# Autodesk Inventor assembly: Ensamblaje de respuesto
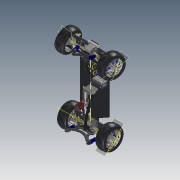
[picture p0: Inventor's stored thumbnail of the model, 180x180]
Saved by Autodesk Inventor 2015 (Build 190159000, 159)
## iProperties
Created: 2015-12-07
Part Number: Ensamblaje de respuesto
Document SubType Name: Assembly
Designer: MIGUEL ANGEL
Author: MIGUEL ANGEL
## Documents named in this file (59)
- C:\Users\MIGUEL ANGEL\Desktop\COCHE\Ensamblaje de respuesto.iam
- C:\Users\MIGUEL ANGEL\Desktop\COCHE\chasis.ipt
- C:\Users\MIGUEL ANGEL\Desktop\COCHE\estructura para ejes ruedas.ipt
- C:\Users\MIGUEL ANGEL\Desktop\COCHE\Pieza direccion.ipt
- C:\Users\MIGUEL ANGEL\Desktop\COCHE\pieza 2 direccion.ipt
- C:\Users\MIGUEL ANGEL\Desktop\COCHE\pieza de chasis.ipt
- C:\Users\MIGUEL ANGEL\Desktop\COCHE\pieza plastico.ipt
- C:\Users\MIGUEL ANGEL\Desktop\COCHE\rotula-eje.ipt
- C:\Users\MIGUEL ANGEL\Desktop\COCHE\pivote de dirección 1.iam
- C:\Users\MIGUEL ANGEL\Desktop\COCHE\tapeta.ipt
- C:\Users\MIGUEL ANGEL\Desktop\COCHE\pieza eje rueda.ipt
- C:\Users\MIGUEL ANGEL\Desktop\COCHE\caja parte 1.ipt
- C:\Users\MIGUEL ANGEL\Desktop\COCHE\pieza del eje.ipt
- C:\Users\MIGUEL ANGEL\Desktop\COCHE\caja de direccion\caja de direccion.iam
- C:\Users\MIGUEL ANGEL\Desktop\COCHE\barra con agarraderas.iam
- C:\Users\MIGUEL ANGEL\Desktop\COCHE\placa direccion 2.ipt
- C:\Users\MIGUEL ANGEL\Desktop\COCHE\pieza articulada de uniones.ipt
- C:\Users\MIGUEL ANGEL\Desktop\COCHE\Ensamblaje de respuesto\Design Accelerator\Conexión por perno1.iam
- C:\Users\MIGUEL ANGEL\Desktop\COCHE\Ensamblaje de respuesto\Design Accelerator\Conexión por perno2.iam
- C:\Users\MIGUEL ANGEL\Desktop\COCHE\barra con agarraderas pequeña.iam
- C:\Users\MIGUEL ANGEL\Desktop\COCHE\eje rueda bueno.ipt
- C:\Users\MIGUEL ANGEL\Desktop\COCHE\tubo para hueso.ipt
- C:\Users\MIGUEL ANGEL\Desktop\COCHE\pieza direccion placa.ipt
- C:\Users\MIGUEL ANGEL\Desktop\COCHE\prueba engranajes.iam
- C:\Users\MIGUEL ANGEL\Desktop\COCHE\eje principal 8 diametro.ipt
- C:\Users\MIGUEL ANGEL\Desktop\COCHE\pieza parte delantera.ipt
- C:\Users\MIGUEL ANGEL\Desktop\COCHE\conexion entre amortiguador y placa.ipt
- C:\Users\MIGUEL ANGEL\Desktop\COCHE\pieza direccion trasera.ipt
- C:\Users\MIGUEL ANGEL\Desktop\COCHE\soporte eje.ipt
- C:\Users\MIGUEL ANGEL\Desktop\COCHE\motor.ipt
- C:\Users\MIGUEL ANGEL\Desktop\COCHE\engranaje 2.iam
- C:\Users\MIGUEL ANGEL\Desktop\COCHE\engranaje 1.iam
- C:\Users\MIGUEL ANGEL\Desktop\COCHE\agarraderas.iam
- C:\Users\MIGUEL ANGEL\Desktop\COCHE\NORMALIZADAS\es-ES\DIN 835\DIN 835 - M6 x 25 - 1.ipt
- C:\Users\MIGUEL ANGEL\Desktop\COCHE\NORMALIZADAS\es-ES\DIN 439-2\DIN 439 - M6 x 1.ipt
- C:\Users\MIGUEL ANGEL\Desktop\COCHE\NORMALIZADAS\es-ES\ANSI B18.22 M\ANSI B18.22M - 6 N.ipt
- C:\Users\MIGUEL ANGEL\Desktop\COCHE\eje rueda bueno trasero.ipt
- C:\Users\MIGUEL ANGEL\Desktop\COCHE\pieza parte trasera.ipt
- C:\Users\MIGUEL ANGEL\Desktop\COCHE\amortiguador.iam
- C:\Users\MIGUEL ANGEL\Desktop\COCHE\armadura.ipt
- C:\Users\MIGUEL ANGEL\Desktop\COCHE\La LLanta.ipt
- C:\Users\MIGUEL ANGEL\Desktop\COCHE\el nuematico.ipt
- C:\Users\MIGUEL ANGEL\Desktop\COCHE\parte motor 2.ipt
- C:\Users\MIGUEL ANGEL\Desktop\COCHE\parte motor 3.ipt
- C:\Users\MIGUEL ANGEL\Desktop\COCHE\caja parte 2 buena.ipt
- C:\Users\MIGUEL ANGEL\Desktop\COCHE\Ensamblaje de respuesto\Design Accelerator\Conexión por perno3.iam
- C:\Users\MIGUEL ANGEL\Desktop\COCHE\Ensamblaje de respuesto\Design Accelerator\Conexión por perno4.iam
- C:\Users\MIGUEL ANGEL\Desktop\COCHE\Ensamblaje de respuesto\Design Accelerator\Conexión por perno5.iam
- C:\Users\MIGUEL ANGEL\Desktop\COCHE\Ensamblaje de respuesto\Design Accelerator\Conexión por perno6.iam
- C:\Users\MIGUEL ANGEL\Desktop\COCHE\Ensamblaje de respuesto\Design Accelerator\Conexión por perno7.iam
- C:\Users\MIGUEL ANGEL\Desktop\COCHE\Ensamblaje de respuesto\Design Accelerator\Conexión por perno8.iam
- C:\Users\MIGUEL ANGEL\Desktop\COCHE\Ensamblaje de respuesto\Design Accelerator\Conexión por perno9.iam
- C:\Users\MIGUEL ANGEL\Desktop\COCHE\Ensamblaje de respuesto\Design Accelerator\Conexión por perno10.iam
- C:\Users\MIGUEL ANGEL\Desktop\COCHE\Ensamblaje de respuesto\Design Accelerator\Conexión por perno12.iam
- C:\Users\MIGUEL ANGEL\Desktop\COCHE\Ensamblaje de respuesto\Design Accelerator\Conexión por perno13.iam
- C:\Users\MIGUEL ANGEL\Desktop\COCHE\Ensamblaje de respuesto\Design Accelerator\Conexión por perno14.iam
- C:\Users\MIGUEL ANGEL\Desktop\COCHE\Ensamblaje de respuesto\Design Accelerator\Conexión por perno15.iam
- C:\Users\MIGUEL ANGEL\Desktop\COCHE\Ensamblaje de respuesto\Design Accelerator\Conexión por perno17.iam
- C:\Users\MIGUEL ANGEL\Desktop\COCHE\Ensamblaje de respuesto\Design Accelerator\Conexión por perno18.iam
## Components (138 placed, 43 different names)
1. chasis:1 — Coincidencia:5, Nivelación:1, Coincidencia:6, Coincidencia:10, Insertar:3, Insertar:4, Coincidencia:27, Coincidencia:28, Nivelación:6, Coincidencia:58, Coincidencia:59, Coincidencia:60, Coincidencia:87, Coincidencia:88, Coincidencia:89, Coincidencia:95, Coincidencia:96, Coincidencia:97, Coincidencia:140, Coincidencia:141, Coincidencia:142, Ángulo:21, Coincidencia:221, Coincidencia:225, Ángulo:25, Coincidencia:267, Coincidencia:269
2. estructura para ejes ruedas:1 — Coincidencia:7, Coincidencia:8, Coincidencia:11, Coincidencia:108, Coincidencia:109, Coincidencia:209
3. pieza de chasis:1 — Coincidencia:5, Nivelación:1, Coincidencia:6, Coincidencia:7, Insertar:1, Ángulo:1, Coincidencia:16, Insertar:2, Ángulo:2
4. pieza plastico:1 — Insertar:1, Ángulo:1, Coincidencia:8
5. rotula-eje:1 — Nivelación:17, Coincidencia:233, Coincidencia:234, Coincidencia:236
6. pieza de chasis:2 — Coincidencia:10, Coincidencia:11
7. pivote de dirección 1:1 [sub-assembly] — Insertar:3, Coincidencia:54, Coincidencia:55, Insertar:13, Coincidencia:68
8. pivote de dirección 1:2 [sub-assembly] — Insertar:4, Coincidencia:52, Coincidencia:53, Coincidencia:69, Coincidencia:70, Coincidencia:205, Ángulo:25
9. estructura para ejes ruedas:2 — Coincidencia:16, Coincidencia:17, Coincidencia:128, Coincidencia:129, Coincidencia:187
10. pieza plastico:2 — Insertar:2, Ángulo:2, Coincidencia:17
11. rotula-eje:2 — Coincidencia:62, Coincidencia:63, Nivelación:18, Coincidencia:245
12. estructura para ejes ruedas:3 — Coincidencia:29, Coincidencia:32, Coincidencia:33, Coincidencia:79, Coincidencia:80, Coincidencia:215
13. estructura para ejes ruedas:4 — Coincidencia:30, Coincidencia:31, Coincidencia:81, Coincidencia:82, Coincidencia:211, Ángulo:21
14. pieza de chasis:3 — Coincidencia:27, Coincidencia:28, Coincidencia:29, Coincidencia:30, Insertar:6, Insertar:7, Nivelación:6, Coincidencia:32
15. pieza plastico:3 — Insertar:6, Coincidencia:31
16. pieza plastico:4 — Insertar:7, Coincidencia:33
17. caja parte 1:1 — Nivelación:8, Coincidencia:77, Coincidencia:95, Coincidencia:96, Coincidencia:97, Coincidencia:102, Insertar:38, Coincidencia:268, Insertar:52, Coincidencia:283, Coincidencia:284, Coincidencia:285, Coincidencia:286
18. placa direccion 2:1 — Coincidencia:50, Coincidencia:51, Coincidencia:56, Coincidencia:57, Coincidencia:203, Coincidencia:204, Coincidencia:205
19. pieza articulada de uniones:1 — Coincidencia:50, Coincidencia:204, Coincidencia:250
20. pieza articulada de uniones:2 — Coincidencia:51, Coincidencia:203, Coincidencia:249
21. Conexión por perno:1 [sub-assembly] — Coincidencia:52, Coincidencia:53, Coincidencia:57
22. Conexión por perno:2 [sub-assembly] — Coincidencia:54, Coincidencia:55, Coincidencia:56
23. barra con agarraderas pequeña:1 [sub-assembly] — Insertar:13, Insertar:15
24. caja de direccion:1 [sub-assembly] — Coincidencia:58, Coincidencia:59, Coincidencia:60, Insertar:15, Coincidencia:275, Coincidencia:276, Coincidencia:277, Coincidencia:278
25. eje rueda bueno:1 — Coincidencia:62, Coincidencia:63, Coincidencia:246, Nivelación:19, Coincidencia:248
26. pieza direccion placa:1 — Coincidencia:68, Coincidencia:69, Coincidencia:70
27. pieza parte delantera:1 — Nivelación:8, Coincidencia:77, Insertar:21, Insertar:22, Coincidencia:102, Coincidencia:116, Coincidencia:123, Coincidencia:133, Coincidencia:158, Nivelación:12, Coincidencia:161, Coincidencia:220, Coincidencia:260
28. conexion entre amortiguador y placa:1 — Insertar:21, Coincidencia:208
29. conexion entre amortiguador y placa:2 — Insertar:22, Coincidencia:186
30. pieza direccion trasera:1 — Coincidencia:79, Coincidencia:80, Coincidencia:83, Coincidencia:84, Coincidencia:170, Coincidencia:171, Coincidencia:178, Nivelación:14, Coincidencia:181, Coincidencia:182, Coincidencia:217
31. pieza direccion trasera:2 — Coincidencia:81, Coincidencia:82, Coincidencia:85, Coincidencia:86, Coincidencia:167, Coincidencia:168, Coincidencia:173, Nivelación:13, Coincidencia:176, Coincidencia:177, Coincidencia:219
32. rotula-eje:3 — Coincidencia:83, Coincidencia:84, Coincidencia:147, Coincidencia:216, Coincidencia:264, Coincidencia:265
33. rotula-eje:4 — Coincidencia:85, Coincidencia:86, Coincidencia:151, Coincidencia:155, Coincidencia:218, Coincidencia:261
34. soporte eje:1 — Coincidencia:87, Coincidencia:88, Coincidencia:89, Coincidencia:99, Insertar:48
35. motor:1 — Coincidencia:253, Coincidencia:254, Insertar:49
36. eje principal 8 diametro:1 — Coincidencia:99, Rotación:1, Coincidencia:198, Coincidencia:200, Ángulo:18, Coincidencia:222, Coincidencia:223, Coincidencia:255, Coincidencia:271, Insertar:53, Ángulo:29
37. engranaje 1:1 [sub-assembly] — Coincidencia:266, Coincidencia:271, Rotación:5, Insertar:53, Ángulo:29
38. engranaje 2:1 [sub-assembly] — Rotación:1, Coincidencia:266, Rotación:5, Coincidencia:273, Ángulo:26, Ángulo:27
39. Pieza direccion:3 — Coincidencia:108, Coincidencia:109, Coincidencia:114, Coincidencia:115, Coincidencia:231, Coincidencia:232, Coincidencia:237
40. DIN 835 M6 x 25:1 — Coincidencia:112, Coincidencia:113, Coincidencia:237, Coincidencia:259
41. DIN 439-2 - reemplazado por DIN EN 24035/28675 M6:1 — Coincidencia:112, Coincidencia:114
42. DIN 439-2 - reemplazado por DIN EN 24035/28675 M6:2 — Coincidencia:113, Coincidencia:115
43. DIN 835 M6 x 25:2 — Coincidencia:116, Coincidencia:119, Coincidencia:120, Coincidencia:121, Coincidencia:122, Coincidencia:258
44. DIN 439-2 - reemplazado por DIN EN 24035/28675 M6:3 — Coincidencia:122, Coincidencia:124
45. DIN 439-2 - reemplazado por DIN EN 24035/28675 M6:4 — Coincidencia:121, Coincidencia:125
46. Arandela plana (Métrico) 6 N:1 — Coincidencia:119, Coincidencia:123, Coincidencia:125
47. Arandela plana (Métrico) 6 N:2 — Coincidencia:120, Coincidencia:124
48. Pieza direccion:4 — Coincidencia:128, Coincidencia:129, Coincidencia:132, Coincidencia:134, Coincidencia:135, Nivelación:9, Coincidencia:138, Coincidencia:139, Coincidencia:243, Coincidencia:244
49. agarraderas:2 [sub-assembly] — Coincidencia:132, Coincidencia:133, Coincidencia:134, Coincidencia:162
50. DIN 835 M6 x 25:3 — Coincidencia:135, Nivelación:9, Coincidencia:136, Coincidencia:137
51. DIN 439-2 - reemplazado por DIN EN 24035/28675 M6:5 — Coincidencia:137, Coincidencia:138
52. DIN 439-2 - reemplazado por DIN EN 24035/28675 M6:6 — Coincidencia:136, Coincidencia:139
53. caja parte 1:2 — Coincidencia:140, Coincidencia:141, Coincidencia:142, Coincidencia:143, Coincidencia:144, Coincidencia:145, Coincidencia:146, Coincidencia:156, Nivelación:11, Coincidencia:157, Coincidencia:270, Coincidencia:293, Coincidencia:294, Coincidencia:299, Coincidencia:300
54. pieza del eje:3 — Coincidencia:143, Coincidencia:145, Coincidencia:152, Ángulo:17, Ángulo:20
55. pieza del eje:4 — Coincidencia:144, Coincidencia:146, Coincidencia:149, Coincidencia:150, Coincidencia:197, Ángulo:19, Ángulo:20
56. eje rueda bueno trasero:1 — Coincidencia:147, Coincidencia:148, Coincidencia:149, Nivelación:10, Coincidencia:265
57. tubo para hueso:3 — Coincidencia:148, Coincidencia:150, Nivelación:10
58. eje rueda bueno trasero:2 — Coincidencia:151, Coincidencia:152, Coincidencia:153, Coincidencia:154, Coincidencia:155
59. tubo para hueso:5 — Coincidencia:153, Ángulo:17, Coincidencia:154
60. pieza parte trasera:1 — Coincidencia:156, Nivelación:11, Coincidencia:157, Coincidencia:169, Coincidencia:172, Nivelación:15, Nivelación:16, Insertar:26, Insertar:29, Insertar:33, Coincidencia:212, Coincidencia:213, Coincidencia:224
61. DIN 835 M6 x 25:4 — Coincidencia:158, Nivelación:12, Coincidencia:159, Coincidencia:160, Coincidencia:163, Coincidencia:164
62. Arandela plana (Métrico) 6 N:3 — Coincidencia:159, Coincidencia:161, Coincidencia:165
63. Arandela plana (Métrico) 6 N:4 — Coincidencia:160, Coincidencia:162, Coincidencia:166
64. DIN 439-2 - reemplazado por DIN EN 24035/28675 M6:7 — Coincidencia:163, Coincidencia:165
65. DIN 439-2 - reemplazado por DIN EN 24035/28675 M6:8 — Coincidencia:164, Coincidencia:166
66. agarraderas:3 [sub-assembly] — Coincidencia:167, Coincidencia:168, Coincidencia:169, Coincidencia:183, Insertar:25
67. agarraderas:4 [sub-assembly] — Coincidencia:170, Coincidencia:171, Coincidencia:172, Coincidencia:184, Insertar:30
68. DIN 835 M6 x 25:5 — Coincidencia:173, Nivelación:13, Coincidencia:174, Coincidencia:175
69. DIN 439-2 - reemplazado por DIN EN 24035/28675 M6:9 — Coincidencia:174, Coincidencia:177
70. DIN 439-2 - reemplazado por DIN EN 24035/28675 M6:10 — Coincidencia:175, Coincidencia:176
71. DIN 835 M6 x 25:6 — Coincidencia:178, Nivelación:14, Coincidencia:179, Coincidencia:180
72. DIN 439-2 - reemplazado por DIN EN 24035/28675 M6:11 — Coincidencia:179, Coincidencia:181
73. DIN 439-2 - reemplazado por DIN EN 24035/28675 M6:12 — Coincidencia:180, Coincidencia:182
74. DIN 835 M6 x 25:8 — Coincidencia:183, Nivelación:15
75. DIN 835 M6 x 25:9 — Coincidencia:184, Nivelación:16
76. Arandela plana (Métrico) 6 N:5 — Insertar:25, Insertar:27
77. Arandela plana (Métrico) 6 N:6 — Insertar:26, Insertar:28
78. DIN 439-2 - reemplazado por DIN EN 24035/28675 M6:13 — Insertar:27
79. DIN 439-2 - reemplazado por DIN EN 24035/28675 M6:14 — Insertar:28
80. Arandela plana (Métrico) 6 N:7 — Insertar:29, Insertar:32
81. Arandela plana (Métrico) 6 N:8 — Insertar:30, Insertar:31
82. DIN 439-2 - reemplazado por DIN EN 24035/28675 M6:15 — Insertar:31
83. DIN 439-2 - reemplazado por DIN EN 24035/28675 M6:16 — Insertar:32
84. conexion entre amortiguador y placa:3 — Insertar:33, Coincidencia:210
85. amortiguador:2 [sub-assembly] — Coincidencia:186, Coincidencia:187
86. engranaje 1:2 [sub-assembly] — Coincidencia:198, Coincidencia:199, Coincidencia:200, Ángulo:18, Rotación:4
87. engranaje 2:2 [sub-assembly] — Coincidencia:197, Coincidencia:199, Ángulo:19, Rotación:4
88. amortiguador:3 [sub-assembly] — Coincidencia:208, Coincidencia:209
89. amortiguador:4 [sub-assembly] — Coincidencia:210, Coincidencia:211
90. amortiguador:5 [sub-assembly] — Coincidencia:214, Coincidencia:215
91. conexion entre amortiguador y placa:4 — Coincidencia:212, Coincidencia:213, Coincidencia:214
92. pieza eje rueda:3 — Coincidencia:216, Coincidencia:217, Insertar:35
93. tapeta:4 — Insertar:35, Insertar:51
94. pieza eje rueda:4 — Coincidencia:218, Coincidencia:219, Insertar:36
95. tapeta:5 — Insertar:36, Insertar:50
96. armadura:1 — Coincidencia:220, Coincidencia:221, Coincidencia:222
97. armadura:2 — Coincidencia:223, Coincidencia:224, Coincidencia:225
98. pieza 2 direccion:3 — Coincidencia:231, Coincidencia:232, Nivelación:17, Coincidencia:233, Insertar:40, Insertar:41
99. eje rueda bueno:2 — Coincidencia:234, Coincidencia:236, Coincidencia:240, Coincidencia:242, Coincidencia:272, Ángulo:27
100. tubo para hueso:6 — Coincidencia:240, Coincidencia:242, Coincidencia:274
101. pieza 2 direccion:4 — Coincidencia:243, Coincidencia:244, Nivelación:18, Coincidencia:245, Insertar:39, Insertar:42
102. pieza del eje:6 — Insertar:38, Coincidencia:247, Coincidencia:248, Ángulo:26
103. tubo para hueso:7 — Coincidencia:246, Nivelación:19, Coincidencia:247
104. barra con agarraderas:1 [sub-assembly] — Coincidencia:249, Insertar:39
105. barra con agarraderas:2 [sub-assembly] — Coincidencia:250, Insertar:40
106. pieza eje rueda:5 — Insertar:41, Insertar:45
107. pieza eje rueda:6 — Insertar:42, Insertar:43
108. La LLanta:1 — Insertar:44, Coincidencia:252
109. La LLanta:2 — Insertar:46, Coincidencia:251
110. tapeta:6 — Insertar:43, Insertar:44
111. tapeta:7 — Insertar:45, Insertar:46
112. el nuematico:1 — Coincidencia:251
113. el nuematico:2 — Coincidencia:252
114. parte motor 2:1 — Coincidencia:253, Coincidencia:254, Insertar:47
115. parte motor 3:1 — Insertar:47
116. prueba engranajes:1 [sub-assembly] — Coincidencia:255, Insertar:48, Insertar:49
117. La LLanta:3 — Insertar:50, Coincidencia:256, Coincidencia:261, Coincidencia:262
118. La LLanta:4 — Insertar:51, Coincidencia:257, Coincidencia:263, Coincidencia:264
119. el nuematico:3 — Coincidencia:256, Coincidencia:262
120. el nuematico:4 — Coincidencia:257, Coincidencia:263
121. agarraderas:5 [sub-assembly] — Coincidencia:258, Coincidencia:259, Coincidencia:260
122. caja parte 2 buena:1 — Coincidencia:267, Coincidencia:268, Coincidencia:279, Coincidencia:280, Coincidencia:281, Coincidencia:282, Coincidencia:287, Coincidencia:288, Coincidencia:289, Coincidencia:290
123. caja parte 2 buena:2 — Coincidencia:269, Coincidencia:270, Coincidencia:295, Coincidencia:296, Coincidencia:297, Coincidencia:298, Coincidencia:301, Coincidencia:302, Coincidencia:303, Coincidencia:304
124. pieza del eje:7 — Insertar:52, Coincidencia:272, Coincidencia:273, Coincidencia:274
125. Conexión por perno:3 [sub-assembly] — Coincidencia:275, Coincidencia:276
126. Conexión por perno:4 [sub-assembly] — Coincidencia:277, Coincidencia:278
127. Conexión por perno:5 [sub-assembly] — Coincidencia:279, Coincidencia:280
128. Conexión por perno:6 [sub-assembly] — Coincidencia:281, Coincidencia:282
129. Conexión por perno:7 [sub-assembly] — Coincidencia:283, Coincidencia:284
130. Conexión por perno:8 [sub-assembly] — Coincidencia:285, Coincidencia:286
131. Conexión por perno:9 [sub-assembly] — Coincidencia:287, Coincidencia:288
132. Conexión por perno:10 [sub-assembly] — Coincidencia:289, Coincidencia:290
133. Conexión por perno:12 [sub-assembly] — Coincidencia:293, Coincidencia:294
134. Conexión por perno:13 [sub-assembly] — Coincidencia:295, Coincidencia:296
135. Conexión por perno:14 [sub-assembly] — Coincidencia:297, Coincidencia:298
136. Conexión por perno:15 [sub-assembly] — Coincidencia:299, Coincidencia:300
137. Conexión por perno:16 [sub-assembly] — Coincidencia:301, Coincidencia:302
138. Conexión por perno:17 [sub-assembly] — Coincidencia:303, Coincidencia:304
## Relationships (277: Mate 212, Insert 37, Flush 14, Angle 11, RelateRotation 3)
- Coincidencia:5 [Mate]: chasis:1 ↔ pieza de chasis:1
- Nivelación:1 [Flush]: chasis:1 ↔ pieza de chasis:1
- Coincidencia:6 [Mate] (0.5 mm): chasis:1 ↔ pieza de chasis:1
- Coincidencia:7 [Mate]: estructura para ejes ruedas:1 ↔ pieza de chasis:1
- Insertar:1: pieza de chasis:1 ↔ pieza plastico:1
- Ángulo:1 [Angle] (0 deg): pieza de chasis:1 ↔ pieza plastico:1
- Coincidencia:8 [Mate]: estructura para ejes ruedas:1 ↔ pieza plastico:1
- Coincidencia:10 [Mate]: chasis:1 ↔ pieza de chasis:2
- Coincidencia:11 [Mate]: estructura para ejes ruedas:1 ↔ pieza de chasis:2
- Coincidencia:16 [Mate]: pieza de chasis:1 ↔ estructura para ejes ruedas:2
- Insertar:2: pieza de chasis:1 ↔ pieza plastico:2
- Ángulo:2 [Angle] (0 deg): pieza de chasis:1 ↔ pieza plastico:2
- Coincidencia:17 [Mate]: estructura para ejes ruedas:2 ↔ pieza plastico:2
- Insertar:3: chasis:1 ↔ pivote de dirección 1:1
- Insertar:4: chasis:1 ↔ pivote de dirección 1:2
- Coincidencia:27 [Mate]: chasis:1 ↔ pieza de chasis:3
- Coincidencia:28 [Mate] (0.5 mm): chasis:1 ↔ pieza de chasis:3
- Coincidencia:29 [Mate]: estructura para ejes ruedas:3 ↔ pieza de chasis:3
- Coincidencia:30 [Mate]: estructura para ejes ruedas:4 ↔ pieza de chasis:3
- Insertar:6: pieza de chasis:3 ↔ pieza plastico:3
- Insertar:7: pieza de chasis:3 ↔ pieza plastico:4
- Nivelación:6 [Flush]: chasis:1 ↔ pieza de chasis:3
- Coincidencia:31 [Mate]: estructura para ejes ruedas:4 ↔ pieza plastico:3
- Coincidencia:32 [Mate]: estructura para ejes ruedas:3 ↔ pieza de chasis:3
- Coincidencia:33 [Mate]: estructura para ejes ruedas:3 ↔ pieza plastico:4
- Coincidencia:50 [Mate]: placa direccion 2:1 ↔ pieza articulada de uniones:1
- Coincidencia:51 [Mate]: placa direccion 2:1 ↔ pieza articulada de uniones:2
- Coincidencia:52 [Mate]: pivote de dirección 1:2 ↔ Conexión por perno:1
- Coincidencia:53 [Mate]: pivote de dirección 1:2 ↔ Conexión por perno:1
- Coincidencia:54 [Mate]: pivote de dirección 1:1 ↔ Conexión por perno:2
- Coincidencia:55 [Mate]: pivote de dirección 1:1 ↔ Conexión por perno:2
- Coincidencia:56 [Mate]: placa direccion 2:1 ↔ Conexión por perno:2
- Coincidencia:57 [Mate]: placa direccion 2:1 ↔ Conexión por perno:1
- Insertar:13: pivote de dirección 1:1 ↔ barra con agarraderas pequeña:1
- Coincidencia:58 [Mate]: chasis:1 ↔ caja de direccion:1
- Coincidencia:59 [Mate]: chasis:1 ↔ caja de direccion:1
- Coincidencia:60 [Mate]: chasis:1 ↔ caja de direccion:1
- Insertar:15: barra con agarraderas pequeña:1 ↔ caja de direccion:1
- Coincidencia:62 [Mate]: rotula-eje:2 ↔ eje rueda bueno:1
- Coincidencia:63 [Mate]: rotula-eje:2 ↔ eje rueda bueno:1
- Coincidencia:68 [Mate]: pivote de dirección 1:1 ↔ pieza direccion placa:1
- Coincidencia:69 [Mate]: pivote de dirección 1:2 ↔ pieza direccion placa:1
- Coincidencia:70 [Mate]: pivote de dirección 1:2 ↔ pieza direccion placa:1
- Nivelación:8 [Flush] (-5 mm): caja parte 1:1 ↔ pieza parte delantera:1
- Coincidencia:77 [Mate]: caja parte 1:1 ↔ pieza parte delantera:1
- Insertar:21: pieza parte delantera:1 ↔ conexion entre amortiguador y placa:1
- Insertar:22: pieza parte delantera:1 ↔ conexion entre amortiguador y placa:2
- Coincidencia:79 [Mate]: estructura para ejes ruedas:3 ↔ pieza direccion trasera:1
- Coincidencia:80 [Mate]: estructura para ejes ruedas:3 ↔ pieza direccion trasera:1
- Coincidencia:81 [Mate]: estructura para ejes ruedas:4 ↔ pieza direccion trasera:2
- Coincidencia:82 [Mate]: estructura para ejes ruedas:4 ↔ pieza direccion trasera:2
- Coincidencia:83 [Mate]: pieza direccion trasera:1 ↔ rotula-eje:3
- Coincidencia:84 [Mate]: pieza direccion trasera:1 ↔ rotula-eje:3
- Coincidencia:85 [Mate]: pieza direccion trasera:2 ↔ rotula-eje:4
- Coincidencia:86 [Mate]: pieza direccion trasera:2 ↔ rotula-eje:4
- Coincidencia:87 [Mate]: chasis:1 ↔ soporte eje:1
- Coincidencia:88 [Mate]: chasis:1 ↔ soporte eje:1
- Coincidencia:89 [Mate]: chasis:1 ↔ soporte eje:1
- Coincidencia:95 [Mate]: chasis:1 ↔ caja parte 1:1
- Coincidencia:96 [Mate]: chasis:1 ↔ caja parte 1:1
- Coincidencia:97 [Mate]: chasis:1 ↔ caja parte 1:1
- Coincidencia:99 [Mate]: soporte eje:1 ↔ eje principal 8 diametro:1
- Coincidencia:102 [Mate]: caja parte 1:1 ↔ pieza parte delantera:1
- Rotación:1 [RelateRotation] (0.2979 ul): eje principal 8 diametro:1 ↔ engranaje 2:1
- Coincidencia:108 [Mate]: estructura para ejes ruedas:1 ↔ Pieza direccion:3
- Coincidencia:109 [Mate]: estructura para ejes ruedas:1 ↔ Pieza direccion:3
- Coincidencia:112 [Mate]: DIN 835 M6 x 25:1 ↔ DIN 439-2 - reemplazado por DIN EN 24035/28675 M6:1
- Coincidencia:113 [Mate]: DIN 835 M6 x 25:1 ↔ DIN 439-2 - reemplazado por DIN EN 24035/28675 M6:2
- Coincidencia:114 [Mate]: Pieza direccion:3 ↔ DIN 439-2 - reemplazado por DIN EN 24035/28675 M6:1
- Coincidencia:115 [Mate]: Pieza direccion:3 ↔ DIN 439-2 - reemplazado por DIN EN 24035/28675 M6:2
- Coincidencia:116 [Mate]: pieza parte delantera:1 ↔ DIN 835 M6 x 25:2
- Coincidencia:119 [Mate]: DIN 835 M6 x 25:2 ↔ Arandela plana (Métrico) 6 N:1
- Coincidencia:120 [Mate]: DIN 835 M6 x 25:2 ↔ Arandela plana (Métrico) 6 N:2
- Coincidencia:121 [Mate]: DIN 835 M6 x 25:2 ↔ DIN 439-2 - reemplazado por DIN EN 24035/28675 M6:4
- Coincidencia:122 [Mate]: DIN 835 M6 x 25:2 ↔ DIN 439-2 - reemplazado por DIN EN 24035/28675 M6:3
- Coincidencia:123 [Mate]: pieza parte delantera:1 ↔ Arandela plana (Métrico) 6 N:1
- Coincidencia:124 [Mate]: DIN 439-2 - reemplazado por DIN EN 24035/28675 M6:3 ↔ Arandela plana (Métrico) 6 N:2
- Coincidencia:125 [Mate]: DIN 439-2 - reemplazado por DIN EN 24035/28675 M6:4 ↔ Arandela plana (Métrico) 6 N:1
- Coincidencia:128 [Mate]: estructura para ejes ruedas:2 ↔ Pieza direccion:4
- Coincidencia:129 [Mate]: estructura para ejes ruedas:2 ↔ Pieza direccion:4
- Coincidencia:132 [Mate]: Pieza direccion:4 ↔ agarraderas:2
- Coincidencia:133 [Mate]: pieza parte delantera:1 ↔ agarraderas:2
- Coincidencia:134 [Mate] (2.5 mm): Pieza direccion:4 ↔ agarraderas:2
- Coincidencia:135 [Mate]: Pieza direccion:4 ↔ DIN 835 M6 x 25:3
- Nivelación:9 [Flush] (5 mm): Pieza direccion:4 ↔ DIN 835 M6 x 25:3
- Coincidencia:136 [Mate]: DIN 835 M6 x 25:3 ↔ DIN 439-2 - reemplazado por DIN EN 24035/28675 M6:6
- Coincidencia:137 [Mate]: DIN 835 M6 x 25:3 ↔ DIN 439-2 - reemplazado por DIN EN 24035/28675 M6:5
- Coincidencia:138 [Mate]: Pieza direccion:4 ↔ DIN 439-2 - reemplazado por DIN EN 24035/28675 M6:5
- Coincidencia:139 [Mate]: Pieza direccion:4 ↔ DIN 439-2 - reemplazado por DIN EN 24035/28675 M6:6
- Coincidencia:140 [Mate]: chasis:1 ↔ caja parte 1:2
- Coincidencia:141 [Mate] (1.2 mm): chasis:1 ↔ caja parte 1:2
- Coincidencia:142 [Mate]: chasis:1 ↔ caja parte 1:2
- Coincidencia:143 [Mate]: caja parte 1:2 ↔ pieza del eje:3
- Coincidencia:144 [Mate]: caja parte 1:2 ↔ pieza del eje:4
- Coincidencia:145 [Mate]: caja parte 1:2 ↔ pieza del eje:3
- Coincidencia:146 [Mate]: caja parte 1:2 ↔ pieza del eje:4
- Coincidencia:147 [Mate]: rotula-eje:3 ↔ eje rueda bueno trasero:1
- Coincidencia:148 [Mate]: eje rueda bueno trasero:1 ↔ tubo para hueso:3
- Coincidencia:149 [Mate]: pieza del eje:4 ↔ eje rueda bueno trasero:1
- Coincidencia:150 [Mate]: pieza del eje:4 ↔ tubo para hueso:3
- Coincidencia:151 [Mate]: rotula-eje:4 ↔ eje rueda bueno trasero:2
- Nivelación:10 [Flush] (-15 mm): eje rueda bueno trasero:1 ↔ tubo para hueso:3
- Coincidencia:152 [Mate]: pieza del eje:3 ↔ eje rueda bueno trasero:2
- Coincidencia:153 [Mate]: eje rueda bueno trasero:2 ↔ tubo para hueso:5
- Ángulo:17 [Angle] (0 deg): pieza del eje:3 ↔ tubo para hueso:5
- Coincidencia:154 [Mate] (-15 mm): eje rueda bueno trasero:2 ↔ tubo para hueso:5
- Coincidencia:155 [Mate]: rotula-eje:4 ↔ eje rueda bueno trasero:2
- Coincidencia:156 [Mate]: caja parte 1:2 ↔ pieza parte trasera:1
- Nivelación:11 [Flush] (5 mm): caja parte 1:2 ↔ pieza parte trasera:1
- Coincidencia:157 [Mate]: caja parte 1:2 ↔ pieza parte trasera:1
- Coincidencia:158 [Mate]: pieza parte delantera:1 ↔ DIN 835 M6 x 25:4
- Nivelación:12 [Flush] (-10 mm): pieza parte delantera:1 ↔ DIN 835 M6 x 25:4
- Coincidencia:159 [Mate]: DIN 835 M6 x 25:4 ↔ Arandela plana (Métrico) 6 N:3
- Coincidencia:160 [Mate]: DIN 835 M6 x 25:4 ↔ Arandela plana (Métrico) 6 N:4
- Coincidencia:161 [Mate]: pieza parte delantera:1 ↔ Arandela plana (Métrico) 6 N:3
- Coincidencia:162 [Mate]: agarraderas:2 ↔ Arandela plana (Métrico) 6 N:4
- Coincidencia:163 [Mate]: DIN 835 M6 x 25:4 ↔ DIN 439-2 - reemplazado por DIN EN 24035/28675 M6:7
- Coincidencia:164 [Mate]: DIN 835 M6 x 25:4 ↔ DIN 439-2 - reemplazado por DIN EN 24035/28675 M6:8
- Coincidencia:165 [Mate]: Arandela plana (Métrico) 6 N:3 ↔ DIN 439-2 - reemplazado por DIN EN 24035/28675 M6:7
- Coincidencia:166 [Mate]: Arandela plana (Métrico) 6 N:4 ↔ DIN 439-2 - reemplazado por DIN EN 24035/28675 M6:8
- Coincidencia:167 [Mate]: pieza direccion trasera:2 ↔ agarraderas:3
- Coincidencia:168 [Mate] (1 mm): pieza direccion trasera:2 ↔ agarraderas:3
- Coincidencia:169 [Mate]: pieza parte trasera:1 ↔ agarraderas:3
- Coincidencia:170 [Mate]: pieza direccion trasera:1 ↔ agarraderas:4
- Coincidencia:171 [Mate] (1 mm): pieza direccion trasera:1 ↔ agarraderas:4
- Coincidencia:172 [Mate]: pieza parte trasera:1 ↔ agarraderas:4
- Coincidencia:173 [Mate]: pieza direccion trasera:2 ↔ DIN 835 M6 x 25:5
- Nivelación:13 [Flush] (5 mm): pieza direccion trasera:2 ↔ DIN 835 M6 x 25:5
- Coincidencia:174 [Mate]: DIN 835 M6 x 25:5 ↔ DIN 439-2 - reemplazado por DIN EN 24035/28675 M6:9
- Coincidencia:175 [Mate]: DIN 835 M6 x 25:5 ↔ DIN 439-2 - reemplazado por DIN EN 24035/28675 M6:10
- Coincidencia:176 [Mate]: pieza direccion trasera:2 ↔ DIN 439-2 - reemplazado por DIN EN 24035/28675 M6:10
- Coincidencia:177 [Mate]: pieza direccion trasera:2 ↔ DIN 439-2 - reemplazado por DIN EN 24035/28675 M6:9
- Coincidencia:178 [Mate]: pieza direccion trasera:1 ↔ DIN 835 M6 x 25:6
- Nivelación:14 [Flush] (5 mm): pieza direccion trasera:1 ↔ DIN 835 M6 x 25:6
- Coincidencia:179 [Mate]: DIN 835 M6 x 25:6 ↔ DIN 439-2 - reemplazado por DIN EN 24035/28675 M6:11
- Coincidencia:180 [Mate]: DIN 835 M6 x 25:6 ↔ DIN 439-2 - reemplazado por DIN EN 24035/28675 M6:12
- Coincidencia:181 [Mate]: pieza direccion trasera:1 ↔ DIN 439-2 - reemplazado por DIN EN 24035/28675 M6:11
- Coincidencia:182 [Mate]: pieza direccion trasera:1 ↔ DIN 439-2 - reemplazado por DIN EN 24035/28675 M6:12
- Coincidencia:183 [Mate]: agarraderas:3 ↔ DIN 835 M6 x 25:8
- Nivelación:15 [Flush] (-8 mm): pieza parte trasera:1 ↔ DIN 835 M6 x 25:8
- Coincidencia:184 [Mate]: agarraderas:4 ↔ DIN 835 M6 x 25:9
- Nivelación:16 [Flush] (8 mm): pieza parte trasera:1 ↔ DIN 835 M6 x 25:9
- Insertar:25: agarraderas:3 ↔ Arandela plana (Métrico) 6 N:5
- Insertar:26: pieza parte trasera:1 ↔ Arandela plana (Métrico) 6 N:6
- Insertar:27: Arandela plana (Métrico) 6 N:5 ↔ DIN 439-2 - reemplazado por DIN EN 24035/28675 M6:13
- Insertar:28: Arandela plana (Métrico) 6 N:6 ↔ DIN 439-2 - reemplazado por DIN EN 24035/28675 M6:14
- Insertar:29: pieza parte trasera:1 ↔ Arandela plana (Métrico) 6 N:7
- Insertar:30: agarraderas:4 ↔ Arandela plana (Métrico) 6 N:8
- Insertar:31: Arandela plana (Métrico) 6 N:8 ↔ DIN 439-2 - reemplazado por DIN EN 24035/28675 M6:15
- Insertar:32: Arandela plana (Métrico) 6 N:7 ↔ DIN 439-2 - reemplazado por DIN EN 24035/28675 M6:16
- Insertar:33: pieza parte trasera:1 ↔ conexion entre amortiguador y placa:3
- Coincidencia:186 [Mate]: conexion entre amortiguador y placa:2 ↔ amortiguador:2
- Coincidencia:187 [Mate]: estructura para ejes ruedas:2 ↔ amortiguador:2
- Coincidencia:197 [Mate]: pieza del eje:4 ↔ engranaje 2:2
- Coincidencia:198 [Mate]: eje principal 8 diametro:1 ↔ engranaje 1:2
- Coincidencia:199 [Mate]: engranaje 1:2 ↔ engranaje 2:2
- Coincidencia:200 [Mate]: eje principal 8 diametro:1 ↔ engranaje 1:2
- Ángulo:18 [Angle] (0 deg): eje principal 8 diametro:1 ↔ engranaje 1:2
- Ángulo:19 [Angle] (0 deg): pieza del eje:4 ↔ engranaje 2:2
- Ángulo:20 [Angle] (0 deg): pieza del eje:3 ↔ pieza del eje:4
- Coincidencia:203 [Mate]: placa direccion 2:1 ↔ pieza articulada de uniones:2
- Coincidencia:204 [Mate]: placa direccion 2:1 ↔ pieza articulada de uniones:1
- Coincidencia:205 [Mate]: pivote de dirección 1:2 ↔ placa direccion 2:1
- Coincidencia:208 [Mate]: conexion entre amortiguador y placa:1 ↔ amortiguador:3
- Coincidencia:209 [Mate]: estructura para ejes ruedas:1 ↔ amortiguador:3
- Coincidencia:210 [Mate]: conexion entre amortiguador y placa:3 ↔ amortiguador:4
- Coincidencia:211 [Mate]: estructura para ejes ruedas:4 ↔ amortiguador:4
- Coincidencia:212 [Mate]: pieza parte trasera:1 ↔ conexion entre amortiguador y placa:4
- Coincidencia:213 [Mate]: pieza parte trasera:1 ↔ conexion entre amortiguador y placa:4
- Coincidencia:214 [Mate]: amortiguador:5 ↔ conexion entre amortiguador y placa:4
- Coincidencia:215 [Mate]: estructura para ejes ruedas:3 ↔ amortiguador:5
- Ángulo:21 [Angle] (0 deg): chasis:1 ↔ estructura para ejes ruedas:4
- Coincidencia:216 [Mate]: rotula-eje:3 ↔ pieza eje rueda:3
- Coincidencia:217 [Mate]: pieza direccion trasera:1 ↔ pieza eje rueda:3
- Insertar:35: pieza eje rueda:3 ↔ tapeta:4
- Coincidencia:218 [Mate]: rotula-eje:4 ↔ pieza eje rueda:4
- Coincidencia:219 [Mate]: pieza direccion trasera:2 ↔ pieza eje rueda:4
- Insertar:36: pieza eje rueda:4 ↔ tapeta:5
- Coincidencia:220 [Mate]: pieza parte delantera:1 ↔ armadura:1
- Coincidencia:221 [Mate]: chasis:1 ↔ armadura:1
- Coincidencia:222 [Mate]: eje principal 8 diametro:1 ↔ armadura:1
- Coincidencia:223 [Mate]: eje principal 8 diametro:1 ↔ armadura:2
- Coincidencia:224 [Mate]: pieza parte trasera:1 ↔ armadura:2
- Coincidencia:225 [Mate]: chasis:1 ↔ armadura:2
- Coincidencia:231 [Mate]: Pieza direccion:3 ↔ pieza 2 direccion:3
- Coincidencia:232 [Mate] (1 mm): Pieza direccion:3 ↔ pieza 2 direccion:3
- Nivelación:17 [Flush] (-48 mm): rotula-eje:1 ↔ pieza 2 direccion:3
- Coincidencia:233 [Mate]: rotula-eje:1 ↔ pieza 2 direccion:3
- Coincidencia:234 [Mate]: rotula-eje:1 ↔ eje rueda bueno:2
- Coincidencia:236 [Mate]: rotula-eje:1 ↔ eje rueda bueno:2
- Coincidencia:237 [Mate]: Pieza direccion:3 ↔ DIN 835 M6 x 25:1
- Coincidencia:240 [Mate]: eje rueda bueno:2 ↔ tubo para hueso:6
- Coincidencia:242 [Mate] (-15.778 mm): eje rueda bueno:2 ↔ tubo para hueso:6
- Coincidencia:243 [Mate]: Pieza direccion:4 ↔ pieza 2 direccion:4
- Coincidencia:244 [Mate] (1 mm): Pieza direccion:4 ↔ pieza 2 direccion:4
- Nivelación:18 [Flush] (-48 mm): rotula-eje:2 ↔ pieza 2 direccion:4
- Coincidencia:245 [Mate]: rotula-eje:2 ↔ pieza 2 direccion:4
- Insertar:38: caja parte 1:1 ↔ pieza del eje:6
- Coincidencia:246 [Mate]: eje rueda bueno:1 ↔ tubo para hueso:7
- Nivelación:19 [Flush] (-15 mm): eje rueda bueno:1 ↔ tubo para hueso:7
- Coincidencia:247 [Mate]: pieza del eje:6 ↔ tubo para hueso:7
- Coincidencia:248 [Mate]: eje rueda bueno:1 ↔ pieza del eje:6
- Coincidencia:249 [Mate]: pieza articulada de uniones:2 ↔ barra con agarraderas:1
- Insertar:39: pieza 2 direccion:4 ↔ barra con agarraderas:1
- Coincidencia:250 [Mate]: pieza articulada de uniones:1 ↔ barra con agarraderas:2
- Insertar:40: pieza 2 direccion:3 ↔ barra con agarraderas:2
- Insertar:41: pieza 2 direccion:3 ↔ pieza eje rueda:5
- Insertar:42: pieza 2 direccion:4 ↔ pieza eje rueda:6
- Ángulo:25 [Angle] (190 deg): chasis:1 ↔ pivote de dirección 1:2
- Insertar:43: pieza eje rueda:6 ↔ tapeta:6
- Insertar:44: La LLanta:1 ↔ tapeta:6
- Insertar:45: pieza eje rueda:5 ↔ tapeta:7
- Insertar:46: La LLanta:2 ↔ tapeta:7
- Coincidencia:251 [Mate]: La LLanta:2 ↔ el nuematico:1
- Coincidencia:252 [Mate]: La LLanta:1 ↔ el nuematico:2
- Coincidencia:253 [Mate]: motor:1 ↔ parte motor 2:1
- Coincidencia:254 [Mate]: motor:1 ↔ parte motor 2:1
- Insertar:47: parte motor 2:1 ↔ parte motor 3:1
- Coincidencia:255 [Mate]: eje principal 8 diametro:1 ↔ prueba engranajes:1
- Insertar:48: soporte eje:1 ↔ prueba engranajes:1
- Insertar:49: motor:1 ↔ prueba engranajes:1
- Insertar:50: tapeta:5 ↔ La LLanta:3
- Insertar:51: tapeta:4 ↔ La LLanta:4
- Coincidencia:256 [Mate]: La LLanta:3 ↔ el nuematico:3
- Coincidencia:257 [Mate]: La LLanta:4 ↔ el nuematico:4
- Coincidencia:258 [Mate]: DIN 835 M6 x 25:2 ↔ agarraderas:5
- Coincidencia:259 [Mate]: DIN 835 M6 x 25:1 ↔ agarraderas:5
- Coincidencia:260 [Mate]: pieza parte delantera:1 ↔ agarraderas:5
- Coincidencia:261 [Mate]: rotula-eje:4 ↔ La LLanta:3
- Coincidencia:262 [Mate]: La LLanta:3 ↔ el nuematico:3
- Coincidencia:263 [Mate]: La LLanta:4 ↔ el nuematico:4
- Coincidencia:264 [Mate]: rotula-eje:3 ↔ La LLanta:4
- Coincidencia:265 [Mate]: rotula-eje:3 ↔ eje rueda bueno trasero:1
- Rotación:4 [RelateRotation] (0.3043 ul): engranaje 1:2 ↔ engranaje 2:2
- Coincidencia:266 [Mate]: engranaje 1:1 ↔ engranaje 2:1
- Coincidencia:267 [Mate]: chasis:1 ↔ caja parte 2 buena:1
- Coincidencia:268 [Mate]: caja parte 1:1 ↔ caja parte 2 buena:1
- Coincidencia:269 [Mate]: chasis:1 ↔ caja parte 2 buena:2
- Coincidencia:270 [Mate]: caja parte 1:2 ↔ caja parte 2 buena:2
- Coincidencia:271 [Mate]: eje principal 8 diametro:1 ↔ engranaje 1:1
- Rotación:5 [RelateRotation] (0.2979 ul): engranaje 1:1 ↔ engranaje 2:1
- Insertar:52: caja parte 1:1 ↔ pieza del eje:7
- Coincidencia:272 [Mate]: eje rueda bueno:2 ↔ pieza del eje:7
- Insertar:53: eje principal 8 diametro:1 ↔ engranaje 1:1
- Coincidencia:273 [Mate]: engranaje 2:1 ↔ pieza del eje:7
- Coincidencia:274 [Mate]: tubo para hueso:6 ↔ pieza del eje:7
- Ángulo:26 [Angle] (0 deg): engranaje 2:1 ↔ pieza del eje:6
- Ángulo:27 [Angle] (0 deg): engranaje 2:1 ↔ eje rueda bueno:2
- Ángulo:29 [Angle] (0 deg): eje principal 8 diametro:1 ↔ engranaje 1:1
- Coincidencia:275 [Mate]: caja de direccion:1 ↔ Conexión por perno:3
- Coincidencia:276 [Mate]: caja de direccion:1 ↔ Conexión por perno:3
- Coincidencia:277 [Mate]: caja de direccion:1 ↔ Conexión por perno:4
- Coincidencia:278 [Mate]: caja de direccion:1 ↔ Conexión por perno:4
- Coincidencia:279 [Mate]: caja parte 2 buena:1 ↔ Conexión por perno:5
- Coincidencia:280 [Mate]: caja parte 2 buena:1 ↔ Conexión por perno:5
- Coincidencia:281 [Mate]: caja parte 2 buena:1 ↔ Conexión por perno:6
- Coincidencia:282 [Mate]: caja parte 2 buena:1 ↔ Conexión por perno:6
- Coincidencia:283 [Mate]: caja parte 1:1 ↔ Conexión por perno:7
- Coincidencia:284 [Mate]: caja parte 1:1 ↔ Conexión por perno:7
- Coincidencia:285 [Mate]: caja parte 1:1 ↔ Conexión por perno:8
- Coincidencia:286 [Mate]: caja parte 1:1 ↔ Conexión por perno:8
- Coincidencia:287 [Mate]: caja parte 2 buena:1 ↔ Conexión por perno:9
- Coincidencia:288 [Mate]: caja parte 2 buena:1 ↔ Conexión por perno:9
- Coincidencia:289 [Mate]: caja parte 2 buena:1 ↔ Conexión por perno:10
- Coincidencia:290 [Mate]: caja parte 2 buena:1 ↔ Conexión por perno:10
- Coincidencia:293 [Mate]: caja parte 1:2 ↔ Conexión por perno:12
- Coincidencia:294 [Mate]: caja parte 1:2 ↔ Conexión por perno:12
- Coincidencia:295 [Mate]: caja parte 2 buena:2 ↔ Conexión por perno:13
- Coincidencia:296 [Mate]: caja parte 2 buena:2 ↔ Conexión por perno:13
- Coincidencia:297 [Mate]: caja parte 2 buena:2 ↔ Conexión por perno:14
- Coincidencia:298 [Mate]: caja parte 2 buena:2 ↔ Conexión por perno:14
- Coincidencia:299 [Mate]: caja parte 1:2 ↔ Conexión por perno:15
- Coincidencia:300 [Mate]: caja parte 1:2 ↔ Conexión por perno:15
- Coincidencia:301 [Mate]: caja parte 2 buena:2 ↔ Conexión por perno:16
- Coincidencia:302 [Mate]: caja parte 2 buena:2 ↔ Conexión por perno:16
- Coincidencia:303 [Mate]: caja parte 2 buena:2 ↔ Conexión por perno:17
- Coincidencia:304 [Mate]: caja parte 2 buena:2 ↔ Conexión por perno:17
